# Autodesk Inventor assembly: Robot Assembly
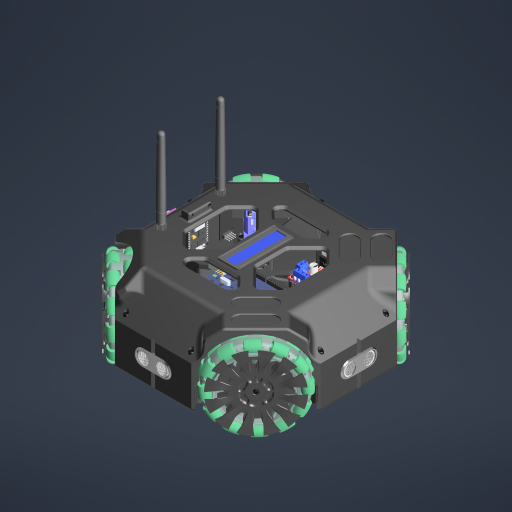
[picture p0: Inventor's stored thumbnail of the model, 512x512]
Saved by Autodesk Inventor 2024 (Build 280153000, 153)
## iProperties
Created: 2025-11-11
Part Number: Robot Assembly
Document SubType Name: Assembly
Designer: Vincent Larson
Author: Vincent Larson
## Documents named in this file (28)
- C:\Users\Vincent Larson\Downloads\Digital Ship Challenge\Digital Ship Challenge Robot\Robot Assembly.iam
- C:\Users\Vincent Larson\Downloads\Digital Ship Challenge\Digital Ship Challenge Robot\Omniwheel\Vex 4in Omniwheel.iam
- C:\Users\Vincent Larson\Downloads\Digital Ship Challenge\Digital Ship Challenge Robot\Adruino Mega\Adruino Mega.ipt
- C:\Users\Vincent Larson\Downloads\Digital Ship Challenge\Digital Ship Challenge Robot\Buck Converter\DC Buck Model.iam
- C:\Users\Vincent Larson\Downloads\Digital Ship Challenge\Digital Ship Challenge Robot\Geared DC Motor\Mini Geared DC Motor _w.iam
- C:\Users\Vincent Larson\Downloads\Digital Ship Challenge\Digital Ship Challenge Robot\GY-BME280-3.3 Sensor\P280, 6-PIN-Version v4.iam
- C:\Users\Vincent Larson\Downloads\Digital Ship Challenge\Digital Ship Challenge Robot\L298N Motor Driver\L298N.ipt
- C:\Users\Vincent Larson\Downloads\Digital Ship Challenge\Digital Ship Challenge Robot\Battery Pack\Battery Pack.ipt
- C:\Users\Vincent Larson\Downloads\Digital Ship Challenge\Digital Ship Challenge Robot\Omniwheel\Omniwheel Mount.ipt
- C:\Users\Vincent Larson\Downloads\Digital Ship Challenge\Digital Ship Challenge Robot\Omniwheel\Omniwheel Cover.ipt
- C:\Users\Vincent Larson\Downloads\Digital Ship Challenge\Digital Ship Challenge Robot\Omniwheel\M3x20 Bolt.ipt
- C:\Users\Vincent Larson\Downloads\Digital Ship Challenge\Digital Ship Challenge Robot\Robot Shell\Robot Shell Front Half.ipt
- C:\Users\Vincent Larson\Downloads\Digital Ship Challenge\Digital Ship Challenge Robot\Robot Shell\Robot Shell Rear Half.ipt
- C:\Users\Vincent Larson\Downloads\Digital Ship Challenge\Digital Ship Challenge Robot\Robot Shell\Robot Shell Bottom Left.ipt
- C:\Users\Vincent Larson\Downloads\Digital Ship Challenge\Digital Ship Challenge Robot\Robot Shell\Robot Shell Bottom Right.ipt
- C:\Users\Vincent Larson\Downloads\Digital Ship Challenge\Digital Ship Challenge Robot\Other Electronics\Metal LED Illuminated Latching 16mm Power Push Button ON-OFF Switch 12V.ipt
- C:\Users\Vincent Larson\Downloads\Digital Ship Challenge\Digital Ship Challenge Robot\Other Electronics\DC Barrel jack.ipt
- C:\Users\Vincent Larson\Downloads\Digital Ship Challenge\Digital Ship Challenge Robot\Other Electronics\USB Type B Socket.ipt
- C:\Users\Vincent Larson\Downloads\Digital Ship Challenge\Digital Ship Challenge Robot\Robot Shell\Axle Holder.ipt
- C:\Users\Vincent Larson\Downloads\Digital Ship Challenge\Digital Ship Challenge Robot\Robot Shell\Arduino & Battery Mount.ipt
- C:\Users\Vincent Larson\Downloads\Digital Ship Challenge\Digital Ship Challenge Robot\NRF24L01L+Antenna\NRF24L01L+Antenna.iam
- C:\Users\Vincent Larson\Downloads\Digital Ship Challenge\Digital Ship Challenge Robot\LCD_I2C_1602\LCD_I2C_1602.ipt
- C:\Users\Vincent Larson\Downloads\Digital Ship Challenge\Digital Ship Challenge Robot\Robot Shell\Robot Shell Top Left.ipt
- C:\Users\Vincent Larson\Downloads\Digital Ship Challenge\Digital Ship Challenge Robot\Ultrasonic sensor\Ultrasonic sensor board.ipt
- C:\Users\Vincent Larson\Downloads\Digital Ship Challenge\Digital Ship Challenge Robot\Ultrasonic sensor\Ultrasonic Sensor.iam
- C:\Users\Vincent Larson\Downloads\Digital Ship Challenge\Digital Ship Challenge Robot\Robot Shell\Robot Shell Top Right.ipt
- C:\Users\Vincent Larson\Downloads\Digital Ship Challenge\Digital Ship Challenge Robot\ESP8266\ESP8266.ipt
- C:\Users\Vincent Larson\Downloads\Digital Ship Challenge\Digital Ship Challenge Robot\Robot Shell\Ultrasonic Sensor Cover.ipt
## Components (80 placed, 27 different names)
1. Adruino Mega:1 — Mate:101
2. DC Buck Model:1 [sub-assembly] — Mate:88
3. P280, 6-PIN-Version v4:1 [sub-assembly] — Mate:125
4. L298N:1 — Mate:91, Mate:92
5. L298N:2 — Mate:90
6. Vex 4in Omniwheel:4 [sub-assembly] — Mate:7, Mate:8, Mate:9, Mate:35, Mate:36
7. Mini Geared DC Motor _w:2 [sub-assembly]
8. Battery Pack:1 — Mate:70
9. Omniwheel Mount:1 — Mate:7, Mate:8, Mate:9
10. Vex 4in Omniwheel:5 [sub-assembly]
11. Mini Geared DC Motor _w:3 [sub-assembly]
12. Omniwheel Mount:2 — Mate:47
13. Vex 4in Omniwheel:6 [sub-assembly]
14. Mini Geared DC Motor _w:4 [sub-assembly]
15. Omniwheel Mount:3 — Mate:48
16. Vex 4in Omniwheel:7 [sub-assembly]
17. Mini Geared DC Motor _w:5 [sub-assembly]
18. Omniwheel Mount:4 — Mate:49
19. Omniwheel Cover:1 — Mate:35, Mate:36, Mate:37, Mate:38
20. M3x20 Bolt:1 — Mate:37, Mate:38
21. Robot Shell Front Half:1 — Mate:39, Flush:8, Flush:9, Flush:11, Flush:12, Mate:53, Mate:73, Mate:74, Mate:75, Mate:76, Mate:107, Mate:108, Mate:112, Mate:114, Mate:126, Mate:127, Mate:128
22. Robot Shell Rear Half:1 — Mate:39, Flush:8, Flush:9, Flush:13, Flush:14, Mate:55, Mate:66, Mate:69, Mate:71, Mate:72, Mate:77, Mate:78, Mate:80, Mate:102, Mate:113
23. Omniwheel Cover:2
24. M3x20 Bolt:2 — Mate:47
25. Omniwheel Cover:3
26. M3x20 Bolt:3 — Mate:48
27. Omniwheel Cover:4
28. M3x20 Bolt:4 — Mate:49
29. Robot Shell Bottom Left:1 — Flush:11, Flush:12, Mate:53, Mate:54, Mate:56, Mate:58, Mate:59, Mate:60, Mate:64, Mate:67, Mate:88, Mate:91, Mate:92, Mate:93, Mate:96, Mate:97
30. Robot Shell Bottom Right:1 — Mate:54, Flush:13, Flush:14, Mate:55, Mate:57, Mate:61, Mate:62, Mate:63, Mate:70, Mate:90, Mate:95, Mate:98, Mate:99
31. M3x20 Bolt:5 — Mate:59, Flush:15, Flush:16
32. M3x20 Bolt:6 — Mate:58, Flush:15, Flush:22, Mate:64
33. M3x20 Bolt:7 — Mate:57, Flush:20, Flush:21
34. M3x20 Bolt:8 — Mate:60, Flush:16, Flush:17
35. M3x20 Bolt:10 — Mate:63, Flush:17, Flush:18
36. M3x20 Bolt:11 — Mate:62, Flush:18, Flush:19
37. M3x20 Bolt:12 — Mate:61, Flush:19, Flush:20
38. M3x20 Bolt:13 — Mate:56, Flush:21, Flush:22
39. Metal LED Illuminated Latching 16mm Power Push Button ON-OFF Switch 12V:1 — Mate:66
40. DC Barrel jack:1 — Mate:67
41. USB Type B Socket:1 — Mate:69
42. Axle Holder:1 — Mate:71, Mate:72, Mate:81, Mate:82, Mate:87
43. Axle Holder:2 — Mate:73, Mate:74, Mate:85, Mate:86
44. Axle Holder:3 — Mate:77, Mate:78, Mate:79
45. Axle Holder:4 — Mate:75, Mate:76, Mate:83, Mate:84
46. M3x20 Bolt:14 — Mate:81, Flush:29
47. M3x20 Bolt:15 — Mate:80, Flush:23, Flush:27
48. M3x20 Bolt:16 — Mate:82, Flush:28, Flush:29, Mate:87
49. M3x20 Bolt:17 — Mate:86, Flush:24, Flush:28
50. M3x20 Bolt:18 — Mate:79, Flush:23
51. M3x20 Bolt:19 — Mate:85, Flush:24, Flush:25
52. M3x20 Bolt:20 — Mate:84, Flush:26, Flush:27
53. M3x20 Bolt:21 — Mate:83, Flush:25, Flush:26
54. Arduino & Battery Mount:1 — Mate:93, Mate:95, Mate:100, Mate:101
55. M3x20 Bolt:22 — Mate:98, Flush:32
56. M3x20 Bolt:23 — Mate:99, Flush:30
57. M3x20 Bolt:24 — Mate:97, Flush:31, Flush:32, Mate:100
58. M3x20 Bolt:25 — Mate:96, Flush:30, Flush:31
59. NRF24L01L+Antenna:1 [sub-assembly] — Flush:33, Flush:34, Mate:110, Mate:111
60. NRF24L01L+Antenna:2 [sub-assembly] — Flush:33, Flush:34
61. LCD_I2C_1602:1 — Flush:39
62. Robot Shell Top Left:1 — Mate:102, Mate:110, Mate:111, Flush:39, Mate:118, Mate:119, Mate:120, Mate:121, Mate:123, Mate:124, Flush:47, Mate:125
63. Ultrasonic sensor board:1 — Mate:107
64. Ultrasonic sensor board:2 — Mate:108
65. Ultrasonic Sensor:1 [sub-assembly] — Mate:112
66. Ultrasonic Sensor:2 [sub-assembly] — Mate:113
67. Ultrasonic Sensor:3 [sub-assembly] — Mate:114
68. M3x20 Bolt:26 — Flush:40, Flush:41
69. M3x20 Bolt:27 — Flush:42, Flush:43
70. M3x20 Bolt:28 — Mate:118, Flush:43, Flush:44
71. M3x20 Bolt:29 — Mate:119, Flush:44, Flush:45
72. M3x20 Bolt:30 — Mate:120, Flush:45, Flush:46
73. M3x20 Bolt:31 — Flush:40
74. M3x20 Bolt:32 — Flush:41, Flush:42
75. M3x20 Bolt:33 — Mate:121, Flush:46, Mate:123
76. Robot Shell Top Right:1 — Mate:124, Flush:47
77. ESP8266:1
78. Ultrasonic Sensor Cover:1 — Mate:128
79. Ultrasonic Sensor Cover:2 — Mate:126
80. Ultrasonic Sensor Cover:3 — Mate:127
## Relationships (128: Mate 93, Flush 35)
- [Mate]: Vex 4in Omniwheel:4 ↔ Mini Geared DC Motor _w:2
- Mate:7: Vex 4in Omniwheel:4 ↔ Omniwheel Mount:1
- Mate:8: Vex 4in Omniwheel:4 ↔ Omniwheel Mount:1
- Mate:9: Vex 4in Omniwheel:4 ↔ Omniwheel Mount:1
- [Mate]: Vex 4in Omniwheel:5 ↔ Mini Geared DC Motor _w:3
- [Mate]: Vex 4in Omniwheel:5 ↔ Omniwheel Mount:2
- [Mate]: Vex 4in Omniwheel:5 ↔ Omniwheel Mount:2
- [Mate]: Vex 4in Omniwheel:5 ↔ Omniwheel Mount:2
- [Mate]: Vex 4in Omniwheel:6 ↔ Mini Geared DC Motor _w:4
- [Mate]: Vex 4in Omniwheel:6 ↔ Omniwheel Mount:3
- [Mate]: Vex 4in Omniwheel:6 ↔ Omniwheel Mount:3
- [Mate]: Vex 4in Omniwheel:6 ↔ Omniwheel Mount:3
- [Mate]: Vex 4in Omniwheel:7 ↔ Mini Geared DC Motor _w:5
- [Mate]: Vex 4in Omniwheel:7 ↔ Omniwheel Mount:4
- [Mate]: Vex 4in Omniwheel:7 ↔ Omniwheel Mount:4
- [Mate]: Vex 4in Omniwheel:7 ↔ Omniwheel Mount:4
- Mate:35: Vex 4in Omniwheel:4 ↔ Omniwheel Cover:1
- Mate:36: Vex 4in Omniwheel:4 ↔ Omniwheel Cover:1
- Mate:37: Omniwheel Cover:1 ↔ M3x20 Bolt:1
- Mate:38: Omniwheel Cover:1 ↔ M3x20 Bolt:1
- Mate:39: Robot Shell Front Half:1 ↔ Robot Shell Rear Half:1
- Flush:8: Robot Shell Front Half:1 ↔ Robot Shell Rear Half:1
- Flush:9: Robot Shell Front Half:1 ↔ Robot Shell Rear Half:1
- [Mate]: Omniwheel Cover:2 ↔ M3x20 Bolt:2
- [Mate]: Omniwheel Cover:2 ↔ M3x20 Bolt:2
- [Mate]: Omniwheel Cover:3 ↔ M3x20 Bolt:3
- [Mate]: Omniwheel Cover:3 ↔ M3x20 Bolt:3
- [Mate]: Omniwheel Cover:4 ↔ M3x20 Bolt:4
- [Mate]: Omniwheel Cover:4 ↔ M3x20 Bolt:4
- Mate:47: Omniwheel Mount:2 ↔ M3x20 Bolt:2
- Mate:48: Omniwheel Mount:3 ↔ M3x20 Bolt:3
- Mate:49: Omniwheel Mount:4 ↔ M3x20 Bolt:4
- Flush:11: Robot Shell Front Half:1 ↔ Robot Shell Bottom Left:1
- Flush:12: Robot Shell Front Half:1 ↔ Robot Shell Bottom Left:1
- Mate:53: Robot Shell Front Half:1 ↔ Robot Shell Bottom Left:1
- Mate:54: Robot Shell Bottom Left:1 ↔ Robot Shell Bottom Right:1
- Flush:13: Robot Shell Rear Half:1 ↔ Robot Shell Bottom Right:1
- Flush:14: Robot Shell Rear Half:1 ↔ Robot Shell Bottom Right:1
- Mate:55: Robot Shell Rear Half:1 ↔ Robot Shell Bottom Right:1
- Mate:56: Robot Shell Bottom Left:1 ↔ M3x20 Bolt:13
- Mate:57: Robot Shell Bottom Right:1 ↔ M3x20 Bolt:7
- Mate:58: Robot Shell Bottom Left:1 ↔ M3x20 Bolt:6
- Mate:59: Robot Shell Bottom Left:1 ↔ M3x20 Bolt:5
- Mate:60: Robot Shell Bottom Left:1 ↔ M3x20 Bolt:8
- Mate:61: Robot Shell Bottom Right:1 ↔ M3x20 Bolt:12
- Mate:62: Robot Shell Bottom Right:1 ↔ M3x20 Bolt:11
- Mate:63: Robot Shell Bottom Right:1 ↔ M3x20 Bolt:10
- Flush:15: M3x20 Bolt:5 ↔ M3x20 Bolt:6
- Flush:16: M3x20 Bolt:5 ↔ M3x20 Bolt:8
- Flush:17: M3x20 Bolt:8 ↔ M3x20 Bolt:10
- Flush:18: M3x20 Bolt:10 ↔ M3x20 Bolt:11
- Flush:19: M3x20 Bolt:11 ↔ M3x20 Bolt:12
- Flush:20: M3x20 Bolt:7 ↔ M3x20 Bolt:12
- Flush:21: M3x20 Bolt:7 ↔ M3x20 Bolt:13
- Flush:22: M3x20 Bolt:6 ↔ M3x20 Bolt:13
- Mate:64: Robot Shell Bottom Left:1 ↔ M3x20 Bolt:6
- Mate:66: Robot Shell Rear Half:1 ↔ Metal LED Illuminated Latching 16mm Power Push Button ON-OFF Switch 12V:1
- Mate:67: Robot Shell Bottom Left:1 ↔ DC Barrel jack:1
- Mate:69: Robot Shell Rear Half:1 ↔ USB Type B Socket:1
- Mate:70: Battery Pack:1 ↔ Robot Shell Bottom Right:1
- Mate:71: Robot Shell Rear Half:1 ↔ Axle Holder:1
- Mate:72: Robot Shell Rear Half:1 ↔ Axle Holder:1
- Mate:73: Robot Shell Front Half:1 ↔ Axle Holder:2
- Mate:74: Robot Shell Front Half:1 ↔ Axle Holder:2
- Mate:75: Robot Shell Front Half:1 ↔ Axle Holder:4
- Mate:76: Robot Shell Front Half:1 ↔ Axle Holder:4
- Mate:77: Robot Shell Rear Half:1 ↔ Axle Holder:3
- Mate:78: Robot Shell Rear Half:1 ↔ Axle Holder:3
- Mate:79: Axle Holder:3 ↔ M3x20 Bolt:18
- Mate:80: Robot Shell Rear Half:1 ↔ M3x20 Bolt:15
- Flush:23: M3x20 Bolt:15 ↔ M3x20 Bolt:18
- Mate:81: Axle Holder:1 ↔ M3x20 Bolt:14
- Mate:82: Axle Holder:1 ↔ M3x20 Bolt:16
- Mate:83: Axle Holder:4 ↔ M3x20 Bolt:21
- Mate:84: Axle Holder:4 ↔ M3x20 Bolt:20
- Mate:85: Axle Holder:2 ↔ M3x20 Bolt:19
- Mate:86: Axle Holder:2 ↔ M3x20 Bolt:17
- Flush:24: M3x20 Bolt:17 ↔ M3x20 Bolt:19
- Flush:25: M3x20 Bolt:19 ↔ M3x20 Bolt:21
- Flush:26: M3x20 Bolt:20 ↔ M3x20 Bolt:21
- Flush:27: M3x20 Bolt:15 ↔ M3x20 Bolt:20
- Flush:28: M3x20 Bolt:16 ↔ M3x20 Bolt:17
- Flush:29: M3x20 Bolt:14 ↔ M3x20 Bolt:16
- Mate:87: Axle Holder:1 ↔ M3x20 Bolt:16
- Mate:88: DC Buck Model:1 ↔ Robot Shell Bottom Left:1
- Mate:90: L298N:2 ↔ Robot Shell Bottom Right:1
- Mate:91: L298N:1 ↔ Robot Shell Bottom Left:1
- Mate:92: L298N:1 ↔ Robot Shell Bottom Left:1
- Mate:93: Robot Shell Bottom Left:1 ↔ Arduino & Battery Mount:1
- Mate:95: Robot Shell Bottom Right:1 ↔ Arduino & Battery Mount:1
- Mate:96: Robot Shell Bottom Left:1 ↔ M3x20 Bolt:25
- Mate:97: Robot Shell Bottom Left:1 ↔ M3x20 Bolt:24
- Mate:98: Robot Shell Bottom Right:1 ↔ M3x20 Bolt:22
- Mate:99: Robot Shell Bottom Right:1 ↔ M3x20 Bolt:23
- Flush:30: M3x20 Bolt:23 ↔ M3x20 Bolt:25
- Flush:31: M3x20 Bolt:24 ↔ M3x20 Bolt:25
- Flush:32: M3x20 Bolt:22 ↔ M3x20 Bolt:24
- Mate:100: Arduino & Battery Mount:1 ↔ M3x20 Bolt:24
- Mate:101: Adruino Mega:1 ↔ Arduino & Battery Mount:1
- Flush:33: NRF24L01L+Antenna:1 ↔ NRF24L01L+Antenna:2
- Flush:34: NRF24L01L+Antenna:1 ↔ NRF24L01L+Antenna:2
- Mate:102: Robot Shell Rear Half:1 ↔ Robot Shell Top Left:1
- Mate:107: Robot Shell Front Half:1 ↔ Ultrasonic sensor board:1
- Mate:108: Robot Shell Front Half:1 ↔ Ultrasonic sensor board:2
- Mate:110: NRF24L01L+Antenna:1 ↔ Robot Shell Top Left:1
- Mate:111: NRF24L01L+Antenna:1 ↔ Robot Shell Top Left:1
- Flush:39: LCD_I2C_1602:1 ↔ Robot Shell Top Left:1
- Mate:112: Robot Shell Front Half:1 ↔ Ultrasonic Sensor:1
- Mate:113: Robot Shell Rear Half:1 ↔ Ultrasonic Sensor:2
- Mate:114: Robot Shell Front Half:1 ↔ Ultrasonic Sensor:3
- Mate:118: Robot Shell Top Left:1 ↔ M3x20 Bolt:28
- Mate:119: Robot Shell Top Left:1 ↔ M3x20 Bolt:29
- Mate:120: Robot Shell Top Left:1 ↔ M3x20 Bolt:30
- Mate:121: Robot Shell Top Left:1 ↔ M3x20 Bolt:33
- Flush:40: M3x20 Bolt:26 ↔ M3x20 Bolt:31
- Flush:41: M3x20 Bolt:26 ↔ M3x20 Bolt:32
- Flush:42: M3x20 Bolt:27 ↔ M3x20 Bolt:32
- Flush:43: M3x20 Bolt:27 ↔ M3x20 Bolt:28
- Flush:44: M3x20 Bolt:28 ↔ M3x20 Bolt:29
- Flush:45: M3x20 Bolt:29 ↔ M3x20 Bolt:30
- Flush:46: M3x20 Bolt:30 ↔ M3x20 Bolt:33
- Mate:123: Robot Shell Top Left:1 ↔ M3x20 Bolt:33
- Mate:124: Robot Shell Top Left:1 ↔ Robot Shell Top Right:1
- Flush:47: Robot Shell Top Left:1 ↔ Robot Shell Top Right:1
- Mate:125: P280, 6-PIN-Version v4:1 ↔ Robot Shell Top Left:1
- Mate:126: Robot Shell Front Half:1 ↔ Ultrasonic Sensor Cover:2
- Mate:127: Robot Shell Front Half:1 ↔ Ultrasonic Sensor Cover:3
- Mate:128: Robot Shell Front Half:1 ↔ Ultrasonic Sensor Cover:1
## Named parameters: d9_d8 = 0 mm, d51_d45 = 0 mm, d52_d46 = 0 mm, d53_d47 = 0 mm, d54_d9_d8 = 0 mm, d55_d45 = 0 mm, d56_d46 = 0 mm, d57_d47 = 0 mm, d58_d9_d8 = 0 mm, d59_d45 = 0 mm, d60_d46 = 0 mm, d61_d47 = 0 mm, d62_d9_d8 = 0 mm, d98_d85 = 0 mm, d99_d86 = 0 mm, d100_d85 = 0 mm, d101_d86 = 0 mm, d102_d85 = 0 mm, d103_d86 = 0 mm
